# Autodesk Inventor assembly: Vex Pulley 18 mm - 42T
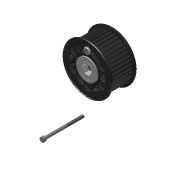
[picture p0: Inventor's stored thumbnail of the model, 180x180]
Saved by Autodesk Inventor 2013 (Build 170138000, 138)
## iProperties
Created: 2013-12-20
Part Number: Vex Pulley 18 mm - 42T
Document SubType Name: Assembly
Designer: Nemo
Author: Nemo
## Documents named in this file (7)
- H:\Nemo\Documents\Robotics\CAD Files\COTS Parts\Pulleys - Vex\Vex Pulley 32 mm - 42T.iam
- H:\Nemo\Documents\Robotics\CAD Files\COTS Parts\Pulleys - Vex\Components\Vex VersaPulley 42T center slice.ipt
- H:\Nemo\Documents\Robotics\CAD Files\COTS Parts\Pulleys - Vex\Components\Vex VersaPulley 42T half.ipt
- H:\Nemo\Documents\Robotics\CAD Files\COTS Parts\Hubs\VersaHub 500 Hex.ipt
- H:\Nemo\Documents\Robotics\CAD Files\COTS Parts\Fasteners\8-32 locknut.ipt
- H:\Nemo\Documents\Robotics\CAD Files\COTS Parts\Bearings - VexPro\Flanged Bearing - 0.5in Hex ID x 1.125in OD.ipt
- H:\Nemo\Documents\Robotics\CAD Files\COTS Parts\Fasteners\8-32 SHCS x1625.ipt
## Components (20 placed, 6 different names)
1. Vex VersaPulley 42T half:1 — Mate:2, Mate:4, Mate:6, Insert:1, Angle:1, Insert:3
2. Vex VersaPulley 42T half:2 — Mate:3, Flush:3, Mate:5, Mate:7, Mate:8, Mate:9
3. VersaHub 500 Hex:1 — Mate:7, Mate:8, Mate:9, Angle:2, Insert:4
4. Flanged Bearing - 0.5in Hex ID x 1.125in OD:1 — Insert:3, Angle:2
5. 8-32 locknut:1 — Insert:1, Angle:1
6. 8-32 SHCS x1625:1 — Insert:4
7. 8-32 locknut:2
8. 8-32 SHCS x1625:2
9. 8-32 locknut:3
10. 8-32 SHCS x1625:3
11. 8-32 locknut:4
12. 8-32 SHCS x1625:4
13. 8-32 locknut:5
14. 8-32 SHCS x1625:5
15. 8-32 locknut:6
16. 8-32 SHCS x1625:6
17. Vex VersaPulley 42T center slice:1 — Mate:1, Flush:1, Flush:2
18. Vex VersaPulley 42T center slice:2 — Mate:6
19. Vex VersaPulley 42T center slice:3 — Mate:5
20. Vex VersaPulley 42T center slice:4
## Component patterns: (2 elements), (6 elements, first: 8-32 locknut:1 + 8-32 SHCS x1625:1), (2 elements, first: Vex VersaPulley 42T center slice:1), Component Pattern 1:2 (2 elements)
## Relationships (17: Mate 9, Flush 3, Insert 3, Angle 2)
- Mate:1: Vex VersaPulley 42T center slice:1
- Flush:1: Vex VersaPulley 42T center slice:1
- Flush:2: Vex VersaPulley 42T center slice:1
- Mate:2: Vex VersaPulley 42T half:1
- Mate:3: Vex VersaPulley 42T half:2
- Mate:4: Vex VersaPulley 42T half:1
- Flush:3: Vex VersaPulley 42T half:2
- Mate:5: Vex VersaPulley 42T half:2 ↔ Vex VersaPulley 42T center slice:3
- Mate:6: Vex VersaPulley 42T half:1 ↔ Vex VersaPulley 42T center slice:2
- Mate:7: Vex VersaPulley 42T half:2 ↔ VersaHub 500 Hex:1
- Mate:8: Vex VersaPulley 42T half:2 ↔ VersaHub 500 Hex:1
- Mate:9: Vex VersaPulley 42T half:2 ↔ VersaHub 500 Hex:1
- Insert:1: Vex VersaPulley 42T half:1 ↔ 8-32 locknut:1
- Angle:1 (0 deg): Vex VersaPulley 42T half:1 ↔ 8-32 locknut:1
- Insert:3: Vex VersaPulley 42T half:1 ↔ Flanged Bearing - 0.5in Hex ID x 1.125in OD:1
- Angle:2 (0 deg): VersaHub 500 Hex:1 ↔ Flanged Bearing - 0.5in Hex ID x 1.125in OD:1
- Insert:4: VersaHub 500 Hex:1 ↔ 8-32 SHCS x1625:1
